# Autodesk Inventor assembly: Recessed Wheels V1.0
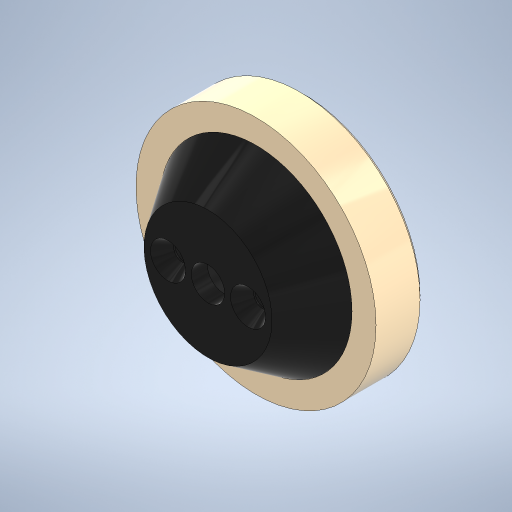
[picture p0: Inventor's stored thumbnail of the model, 512x512]
Saved by Autodesk Inventor 2023.4 (Build 274418000, 418)
## iProperties
Created: 2023-02-06
Part Number: Recessed Wheels V1.0
Document SubType Name: Assembly
Designer: Nathan Cai
Mass: 37.0779 g
Surface Area: 111.741 cm^2
Volume: 16.017 cm^3
Density: 2.31491 g/cm^3
Author: Nathan Cai
## Documents named in this file (4)
- E:\Documents\Inventor\IMchass V3.0\Custom Wheel V1.0\Recessed Wheels V1.0.iam
- E:\Documents\Inventor\IMchass V3.0\Custom Wheel V1.0\Botkit-Hubs\Botkit-Hubs.iam
- E:\Documents\Inventor\IMchass V3.0\Custom Wheel V1.0\Tire Hub.ipt
- E:\Documents\Inventor\IMchass V3.0\Custom Wheel V1.0\Tire.ipt
## Components (3 placed, 3 different names)
1. Botkit-Hubs:1 [sub-assembly] — Mate:1, Mate:2, Mate:3
2. Tire Hub:1 — Mate:1, Mate:2, Mate:3, Mate:4, Mate:5
3. Tire:1 — Mate:4, Mate:5
## Relationships (5: Mate 5)
- Mate:1: Botkit-Hubs:1 ↔ Tire Hub:1
- Mate:2: Botkit-Hubs:1 ↔ Tire Hub:1
- Mate:3: Botkit-Hubs:1 ↔ Tire Hub:1
- Mate:4: Tire Hub:1 ↔ Tire:1
- Mate:5: Tire Hub:1 ↔ Tire:1
